# Autodesk Inventor assembly: Full Assembly
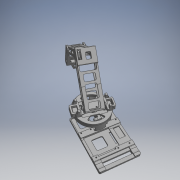
[picture p0: Inventor's stored thumbnail of the model, 180x180]
Saved by Autodesk Inventor 2020.5 (Build 245400000, 400)
## iProperties
Created: 2023-03-27
Part Number: Full Assembly
Document SubType Name: Assembly
Designer: Wes
Author: Wes
## Documents named in this file (8)
- C:\Users\Wes\Documents\Wes Stuff\Programming\Python\CPEN291\P2_L2B_G8\3D Design\Arm Full Assembly.iam
- C:\Users\Wes\Documents\Wes Stuff\Programming\Python\CPEN291\P2_L2B_G8\3D Design\Arm Lower Shortened.iam
- C:\Users\Wes\Documents\Wes Stuff\Programming\Python\CPEN291\P2_L2B_G8\3D Design\Arm Middle.ipt
- C:\Users\Wes\Documents\Wes Stuff\Programming\Python\CPEN291\P2_L2B_G8\3D Design\Arm Upper.ipt
- C:\Users\Wes\Documents\Wes Stuff\Programming\Python\CPEN291\P2_L2B_G8\3D Design\Swivel Top.ipt
- C:\Users\Wes\Documents\Wes Stuff\Programming\Python\CPEN291\P2_L2B_G8\3D Design\Swivel Base.ipt
- C:\Users\Wes\Documents\Wes Stuff\Programming\Python\CPEN291\P2_L2B_G8\3D Design\Base Extension 1.ipt
- C:\Users\Wes\Documents\Wes Stuff\Programming\Python\CPEN291\P2_L2B_G8\3D Design\Base Extension 2.ipt
## Components (7 placed, 7 different names)
1. Arm Lower Shortened:1 [sub-assembly] — Rotational:1, Rotational:3
2. Arm Middle:1 — Rotational:1, Rotational:2
3. Arm Upper:1 — Rotational:2
4. Swivel Top:1 — Rotational:3, Rotational:4
5. Swivel Base:1 — Rotational:4, Mate:1, Mate:2, Flush:1
6. Base Extension 1:1 — Mate:1, Mate:2, Flush:1, Mate:3, Flush:2, Mate:4
7. Base Extension 2:1 — Mate:3, Flush:2, Mate:4
## Relationships (10: RevoluteJoint 4, Mate 4, Flush 2)
- Rotational:1 [RevoluteJoint]: Arm Lower Shortened:1 ↔ Arm Middle:1
- Rotational:2 [RevoluteJoint]: Arm Middle:1 ↔ Arm Upper:1
- Rotational:3 [RevoluteJoint] (18.5 mm): Arm Lower Shortened:1 ↔ Swivel Top:1
- Rotational:4 [RevoluteJoint] (-19.6 mm): Swivel Top:1 ↔ Swivel Base:1
- Mate:1: Swivel Base:1 ↔ Base Extension 1:1
- Mate:2 (0.5 mm): Swivel Base:1 ↔ Base Extension 1:1
- Flush:1: Swivel Base:1 ↔ Base Extension 1:1
- Mate:3: Base Extension 1:1 ↔ Base Extension 2:1
- Flush:2: Base Extension 1:1 ↔ Base Extension 2:1
- Mate:4: Base Extension 1:1 ↔ Base Extension 2:1
